# Autodesk Inventor assembly: Assembly1
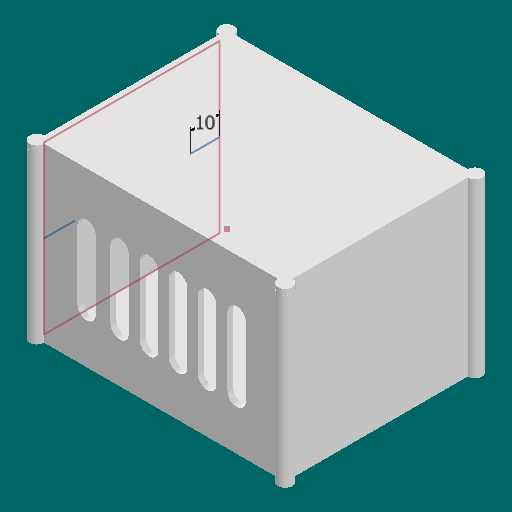
[picture p0: Inventor's stored thumbnail of the model, 512x512]
Saved by Autodesk Inventor 2025.2 (Build 292293000, 293)
## iProperties
Created: 2025-06-02
Part Number: Assembly1
Document SubType Name: Assembly
Designer: ia088
Author: ia088
## Documents named in this file (3)
- C:\Users\ia088\OneDrive\Dokumen\subki\Assembly1.iam
- C:\Users\ia088\OneDrive\Dokumen\Body_Bottom.ipt
- C:\Users\ia088\OneDrive\Dokumen\Part2.ipt
## Components (2 placed, 2 different names)
1. Body_Bottom:1 — Flush:1, Flush:2
2. Part2:1 — Flush:1, Flush:2
## Relationships (2: Flush 2)
- Flush:1: Body_Bottom:1 ↔ Part2:1
- Flush:2: Body_Bottom:1 ↔ Part2:1
